# Autodesk Inventor assembly: Assembly2
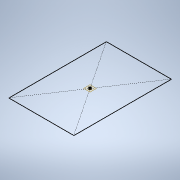
[picture p0: Inventor's stored thumbnail of the model, 180x180]
Saved by Autodesk Inventor 2020 (Build 240168000, 168)
## iProperties
Created: 2021-08-27
Part Number: Assembly2
Document SubType Name: Assembly
Designer: Masato
Author: Masato
## Documents named in this file (1)
- C:\Users\Masato\Desktop\Assembly2.iam
## Relationships (1: Flush 1)
- フラッシュ:1 [Flush]
